# Autodesk Inventor assembly: 0.3rd Lawette - V3.0
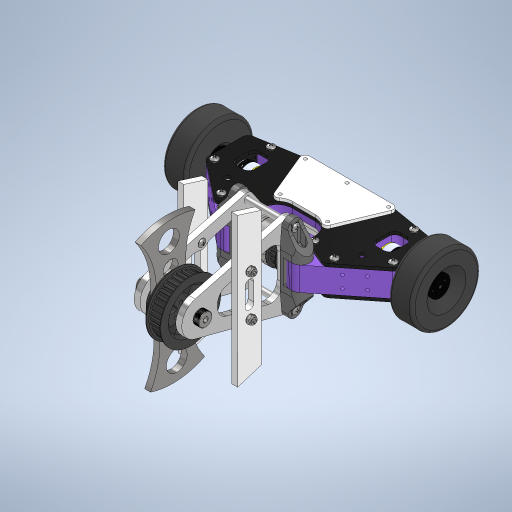
[picture p0: Inventor's stored thumbnail of the model, 512x512]
Saved by Autodesk Inventor 2023 (Build 270158000, 158)
## iProperties
Created: 2022-05-21
Part Number: 0.3rd Lawette - V3.0
Document SubType Name: Assembly
Designer: Nathan Cai
Mass: 1254.41 g
Surface Area: 3808.05 cm^2
Volume: 766.959 cm^3
Density: 1.63556 g/cm^3
Author: Nathan Cai
## Documents named in this file (23)
- E:\Documents\Inventor\0.3rd Lawette - V3.1\0.3rd Lawette - V3.1.iam
- E:\Documents\Inventor\0.3rd Lawette - V3.1\RR Brushless\RR-Brushless-Planetary.iam
- E:\Documents\Inventor\0.3rd Lawette - V3.1\Tattu 4S 650mah\Tattu 650mah 4S.iam
- E:\Documents\Inventor\0.3rd Lawette - V3.1\BL20A.ipt
- E:\Documents\Inventor\0.3rd Lawette - V3.1\Talon 25A ESC.ipt
- E:\Documents\Inventor\0.3rd Lawette - V3.1\Receiver (FrSky RX6R).ipt
- E:\Documents\Inventor\0.3rd Lawette - V3.1\Fingertech Power Switch\Fingertech Mini Power Switch.iam
- E:\Documents\Inventor\0.3rd Lawette - V3.1\Weapon Assembly.iam
- E:\Documents\Inventor\0.3rd Lawette - V3.1\Hubs (Fingertech Twisthub).ipt
- E:\Documents\Inventor\0.3rd Lawette - V3.1\Chassis.ipt
- E:\Documents\Inventor\0.3rd Lawette - V3.1\Tires (Fingertech Foam Wheels).ipt
- E:\Documents\Inventor\0.3rd Lawette - V3.1\Standoff 1.5in.ipt
- E:\Documents\Inventor\0.3rd Lawette - V3.1\Bracket.ipt
- E:\Documents\Inventor\Content Center Files\R2022\en-US\ANSI B18.6.3(27)\ANSI B18.6.3 - 6-32 UNC - 0.625(11).ipt
- E:\Documents\Inventor\0.3rd Lawette - V3.1\Motor Plates.ipt
- E:\Documents\Inventor\0.3rd Lawette - V3.1\Motor Plates - Rear Insert.ipt
- E:\Documents\Inventor\0.3rd Lawette - V3.1\Cover (Inner Bottom).ipt
- E:\Documents\Inventor\0.3rd Lawette - V3.1\Cover (Inner Top).ipt
- E:\Documents\Inventor\0.3rd Lawette - V3.1\Cover (Outer).ipt
- E:\Documents\Inventor\0.3rd Lawette - V3.1\Standoff 1in.ipt
- E:\Documents\Inventor\Content Center Files\R2022\en-US\ANSI B18.6.3(27)\ANSI B18.6.3 - 6-32 UNC - 0.875(11).ipt
- E:\Documents\Inventor\Content Center Files\R2022\en-US\ANSI B18.22.1\ANSI B18.22.1 - No. 6 - narrow - Type B.ipt
- E:\Documents\Inventor\Content Center Files\R2022\en-US\ANSI B18.6.3(27)\ANSI B18.6.3 - 6-32 UNC - 0.5(11).ipt
## Components (84 placed, 22 different names)
1. RR-Brushless-Planetary:1 [sub-assembly] — Mate:1, Mate:4, Mate:7, Flush:4, Mate:27, Mate:147
2. RR-Brushless-Planetary:2 [sub-assembly] — Mate:1, Mate:5, Mate:6, Flush:5, Mate:149
3. Tattu 650mah 4S:1 [sub-assembly] — Mate:15, Flush:9
4. BL20A:1 — Mate:2, Flush:1, Flush:2, Mate:14, Flush:7
5. BL20A:2 — Mate:2, Flush:1, Flush:2, Mate:3, Flush:3, Flush:8
6. Talon 25A ESC:1 — Mate:13, Flush:6, Mate:151
7. Receiver (FrSky RX6R):1 — Mate:3, Flush:3, Flush:8
8. Fingertech Mini Power Switch:1 [sub-assembly] — Flush:12, Mate:26, Mate:150
9. Hubs (Fingertech Twisthub):1 — Mate:4, Mate:7, Mate:8, Mate:11
10. Hubs (Fingertech Twisthub):2 — Mate:5, Mate:6, Mate:9, Mate:155
11. Chassis:1 — Flush:4, Flush:5, Mate:13, Flush:6, Mate:14, Flush:7, Mate:15, Flush:9, Flush:12, Mate:26, Mate:27, Mate:113, Mate:114, Mate:115, Mate:116, Mate:117, Mate:118, Mate:119, Mate:120, Mate:121, Mate:146, Flush:20, Mate:148, Flush:21, Mate:150, Mate:151, Mate:152, Mate:156, Mate:165, Mate:166, Mate:167, Mate:168, Mate:169, Mate:170, Mate:171, Mate:172, Mate:173, Mate:174, Mate:175, Mate:176, Mate:177, Flush:32, Mate:184, Mate:186, Mate:187
12. Tires (Fingertech Foam Wheels):1 — Mate:9, Mate:155
13. Tires (Fingertech Foam Wheels):2 — Mate:8, Mate:11
14. Motor Plates:1 — Mate:113, Mate:114, Mate:115
15. Motor Plates:2 — Mate:116, Mate:117, Mate:118
16. Motor Plates - Rear Insert:1 — Mate:146, Mate:147, Flush:20
17. Motor Plates - Rear Insert:2 — Mate:148, Mate:149, Flush:21
18. Cover (Inner Bottom):1 — Mate:152, Mate:159, Mate:160, Mate:161, Mate:216, Mate:217, Mate:218, Mate:219, Mate:220, Mate:221, Mate:222, Mate:223, Mate:224, Mate:225, Mate:226, Mate:227, Mate:228, Mate:229, Mate:230, Mate:231
19. Cover (Inner Top):1 — Mate:156, Mate:162, Mate:163, Mate:164, Mate:165, Mate:166, Mate:200, Mate:201, Mate:202, Mate:203, Mate:204, Mate:205, Mate:206, Mate:207, Mate:208, Mate:209, Mate:210, Mate:211, Mate:212, Mate:213, Mate:214, Mate:215
20. Cover (Outer):1 — Mate:159, Mate:160, Mate:161
21. Cover (Outer):2 — Mate:162, Mate:163, Mate:164
22. Standoff 1in:1 — Flush:22, Flush:23, Flush:24, Flush:25, Flush:26, Flush:27, Flush:28, Flush:29, Flush:30, Flush:31, Mate:167, Flush:32, Flush:33, Flush:34
23. Standoff 1in:2 — Flush:22, Mate:168
24. Standoff 1in:3 — Flush:25, Mate:175
25. Standoff 1in:4 — Flush:27, Mate:174
26. Standoff 1in:5 — Flush:29, Mate:173
27. Standoff 1in:6 — Flush:23, Mate:177
28. Standoff 1in:7 — Flush:24, Mate:176
29. Standoff 1in:8 — Flush:26, Mate:169
30. Standoff 1in:9 — Flush:28, Mate:170
31. Standoff 1in:10 — Flush:30, Mate:171
32. Standoff 1in:11 — Flush:31, Mate:172
33. Bracket:1 — Mate:178, Mate:179, Mate:180, Mate:185, Mate:196, Mate:197, Mate:198, Mate:199
34. Bracket:2 — Mate:181, Mate:182, Mate:183, Mate:184, Mate:192, Mate:193, Mate:194, Mate:195
35. Standoff 1in:12 — Mate:186, Flush:34
36. Standoff 1in:13 — Mate:187, Flush:33
37. Cross Recessed Truss Head Machine Screw - Type I - Inch No. 6 - 32 - 7/8:1 — Insert:5
38. Plain Washer (Inch) No. 6 - narrow - Type B:1 — Mate:192, Mate:193, Insert:3
39. Cross Recessed Truss Head Machine Screw - Type I - Inch No. 6 - 32 - 7/8:3 — Insert:3
40. Plain Washer (Inch) No. 6 - narrow - Type B:2 — Mate:194, Mate:195, Insert:4
41. Cross Recessed Truss Head Machine Screw - Type I - Inch No. 6 - 32 - 7/8:4 — Insert:4
42. Plain Washer (Inch) No. 6 - narrow - Type B:3 — Mate:196, Mate:197, Insert:5
43. Plain Washer (Inch) No. 6 - narrow - Type B:4 — Mate:198, Mate:199, Insert:6
44. Cross Recessed Truss Head Machine Screw - Type I - Inch No. 6 - 32 - 7/8:5 — Insert:6
45. Plain Washer (Inch) No. 6 - narrow - Type B:5 — Mate:200, Mate:201, Insert:7
46. Cross Recessed Truss Head Machine Screw - Type I - Inch No. 6 - 32 - 1/2:1 — Insert:7
47. Plain Washer (Inch) No. 6 - narrow - Type B:6 — Mate:202, Mate:203, Insert:8
48. Plain Washer (Inch) No. 6 - narrow - Type B:7 — Mate:204, Mate:205, Insert:9
49. Plain Washer (Inch) No. 6 - narrow - Type B:8 — Mate:206, Mate:207, Insert:10
50. Plain Washer (Inch) No. 6 - narrow - Type B:9 — Mate:208, Mate:209, Insert:11
51. Plain Washer (Inch) No. 6 - narrow - Type B:10 — Mate:210, Mate:211, Insert:12
52. Plain Washer (Inch) No. 6 - narrow - Type B:11 — Mate:212, Mate:213, Insert:13
53. Plain Washer (Inch) No. 6 - narrow - Type B:12 — Mate:214, Mate:215, Insert:14
54. Cross Recessed Truss Head Machine Screw - Type I - Inch No. 6 - 32 - 1/2:2 — Insert:8
55. Cross Recessed Truss Head Machine Screw - Type I - Inch No. 6 - 32 - 1/2:3 — Insert:9
56. Cross Recessed Truss Head Machine Screw - Type I - Inch No. 6 - 32 - 1/2:4 — Insert:10
57. Cross Recessed Truss Head Machine Screw - Type I - Inch No. 6 - 32 - 1/2:5 — Insert:11
58. Cross Recessed Truss Head Machine Screw - Type I - Inch No. 6 - 32 - 1/2:6 — Insert:12
59. Cross Recessed Truss Head Machine Screw - Type I - Inch No. 6 - 32 - 1/2:7 — Insert:13
60. Cross Recessed Truss Head Machine Screw - Type I - Inch No. 6 - 32 - 1/2:8 — Insert:14
61. Plain Washer (Inch) No. 6 - narrow - Type B:13 — Mate:216, Mate:217, Insert:15
62. Cross Recessed Truss Head Machine Screw - Type I - Inch No. 6 - 32 - 1/2:9 — Insert:15
63. Plain Washer (Inch) No. 6 - narrow - Type B:14 — Mate:218, Mate:219, Insert:16
64. Plain Washer (Inch) No. 6 - narrow - Type B:15 — Mate:220, Mate:221, Insert:17
65. Plain Washer (Inch) No. 6 - narrow - Type B:16 — Mate:222, Mate:223, Insert:18
66. Plain Washer (Inch) No. 6 - narrow - Type B:17 — Mate:224, Mate:225, Insert:19
67. Plain Washer (Inch) No. 6 - narrow - Type B:18 — Mate:226, Mate:227, Insert:20
68. Plain Washer (Inch) No. 6 - narrow - Type B:19 — Mate:228, Mate:229, Insert:21
69. Plain Washer (Inch) No. 6 - narrow - Type B:20 — Mate:230, Mate:231, Insert:22
70. Cross Recessed Truss Head Machine Screw - Type I - Inch No. 6 - 32 - 1/2:10 — Insert:16
71. Cross Recessed Truss Head Machine Screw - Type I - Inch No. 6 - 32 - 1/2:11 — Insert:17
72. Cross Recessed Truss Head Machine Screw - Type I - Inch No. 6 - 32 - 1/2:12 — Insert:18
73. Cross Recessed Truss Head Machine Screw - Type I - Inch No. 6 - 32 - 1/2:13 — Insert:19
74. Cross Recessed Truss Head Machine Screw - Type I - Inch No. 6 - 32 - 1/2:14 — Insert:20
75. Cross Recessed Truss Head Machine Screw - Type I - Inch No. 6 - 32 - 1/2:15 — Insert:21
76. Cross Recessed Truss Head Machine Screw - Type I - Inch No. 6 - 32 - 1/2:16 — Insert:22
77. Standoff 1.5in:7 — Mate:93, Mate:94, Mate:95, Mate:96, Mate:185
78. Standoff 1.5in:8 — Mate:97, Mate:98, Mate:99, Mate:100
79. Weapon Assembly:1 [sub-assembly] — Mate:178, Mate:179, Mate:180, Mate:181, Mate:182, Mate:183
80. Cross Recessed Truss Head Machine Screw - Type I - Inch No. 6 - 32 - 5/8:1 — Mate:93, Mate:94
81. Cross Recessed Truss Head Machine Screw - Type I - Inch No. 6 - 32 - 5/8:2 — Mate:95, Mate:96
82. Cross Recessed Truss Head Machine Screw - Type I - Inch No. 6 - 32 - 5/8:4 — Mate:99, Mate:100
83. Cross Recessed Truss Head Machine Screw - Type I - Inch No. 6 - 32 - 5/8:3 — Mate:97, Mate:98
84. Weapon Assembly:2 [sub-assembly] — Mate:119, Mate:120, Mate:121
## Relationships (159: Mate 112, Flush 27, Insert 20)
- Mate:1: RR-Brushless-Planetary:1 ↔ RR-Brushless-Planetary:2
- Mate:2: BL20A:1 ↔ BL20A:2
- Flush:1: BL20A:1 ↔ BL20A:2
- Flush:2: BL20A:1 ↔ BL20A:2
- Mate:3: BL20A:2 ↔ Receiver (FrSky RX6R):1
- Flush:3: BL20A:2 ↔ Receiver (FrSky RX6R):1
- Mate:4: RR-Brushless-Planetary:1 ↔ Hubs (Fingertech Twisthub):1
- Mate:5: RR-Brushless-Planetary:2 ↔ Hubs (Fingertech Twisthub):2
- Mate:6: RR-Brushless-Planetary:2 ↔ Hubs (Fingertech Twisthub):2
- Mate:7: RR-Brushless-Planetary:1 ↔ Hubs (Fingertech Twisthub):1
- Mate:8: Hubs (Fingertech Twisthub):1 ↔ Tires (Fingertech Foam Wheels):2
- Mate:9: Hubs (Fingertech Twisthub):2 ↔ Tires (Fingertech Foam Wheels):1
- Mate:11: Hubs (Fingertech Twisthub):1 ↔ Tires (Fingertech Foam Wheels):2
- Flush:4: RR-Brushless-Planetary:1 ↔ Chassis:1
- Flush:5: RR-Brushless-Planetary:2 ↔ Chassis:1
- Mate:13: Talon 25A ESC:1 ↔ Chassis:1
- Flush:6: Talon 25A ESC:1 ↔ Chassis:1
- Mate:14: BL20A:1 ↔ Chassis:1
- Flush:7: BL20A:1 ↔ Chassis:1
- Flush:8: BL20A:2 ↔ Receiver (FrSky RX6R):1
- Mate:15 (3.175 mm): Tattu 650mah 4S:1 ↔ Chassis:1
- Flush:9: Tattu 650mah 4S:1 ↔ Chassis:1
- Flush:12: Fingertech Mini Power Switch:1 ↔ Chassis:1
- [Mate]: Chassis:1 ↔ Standoff 1.5in:8
- [Mate]: Chassis:1 ↔ Standoff 1.5in:7
- Mate:26: Fingertech Mini Power Switch:1 ↔ Chassis:1
- Mate:27: RR-Brushless-Planetary:1 ↔ Chassis:1
- [Flush] (-6.35 mm): Chassis:1 ↔ Standoff 1.5in:8
- [Flush]: Standoff 1.5in:7 ↔ Standoff 1.5in:8
- Mate:93: Standoff 1.5in:7 ↔ Cross Recessed Truss Head Machine Screw - Type I - Inch No. 6 - 32 - 5/8:1
- Mate:94: Standoff 1.5in:7 ↔ Cross Recessed Truss Head Machine Screw - Type I - Inch No. 6 - 32 - 5/8:1
- Mate:95: Standoff 1.5in:7 ↔ Cross Recessed Truss Head Machine Screw - Type I - Inch No. 6 - 32 - 5/8:2
- Mate:96: Standoff 1.5in:7 ↔ Cross Recessed Truss Head Machine Screw - Type I - Inch No. 6 - 32 - 5/8:2
- Mate:97: Standoff 1.5in:8 ↔ Cross Recessed Truss Head Machine Screw - Type I - Inch No. 6 - 32 - 5/8:3
- Mate:98: Standoff 1.5in:8 ↔ Cross Recessed Truss Head Machine Screw - Type I - Inch No. 6 - 32 - 5/8:3
- Mate:99: Standoff 1.5in:8 ↔ Cross Recessed Truss Head Machine Screw - Type I - Inch No. 6 - 32 - 5/8:4
- Mate:100: Standoff 1.5in:8 ↔ Cross Recessed Truss Head Machine Screw - Type I - Inch No. 6 - 32 - 5/8:4
- Mate:113: Chassis:1 ↔ Motor Plates:1
- Mate:114: Chassis:1 ↔ Motor Plates:1
- Mate:115: Chassis:1 ↔ Motor Plates:1
- Mate:116: Chassis:1 ↔ Motor Plates:2
- Mate:117: Chassis:1 ↔ Motor Plates:2
- Mate:118: Chassis:1 ↔ Motor Plates:2
- Mate:119: Chassis:1 ↔ Weapon Assembly:2
- Mate:120: Chassis:1 ↔ Weapon Assembly:2
- Mate:121 (9.525 mm): Chassis:1 ↔ Weapon Assembly:2
- Mate:146: Chassis:1 ↔ Motor Plates - Rear Insert:1
- Mate:147: RR-Brushless-Planetary:1 ↔ Motor Plates - Rear Insert:1
- Flush:20: Chassis:1 ↔ Motor Plates - Rear Insert:1
- Mate:148: Chassis:1 ↔ Motor Plates - Rear Insert:2
- Mate:149: RR-Brushless-Planetary:2 ↔ Motor Plates - Rear Insert:2
- Flush:21: Chassis:1 ↔ Motor Plates - Rear Insert:2
- Mate:150: Fingertech Mini Power Switch:1 ↔ Chassis:1
- Mate:151: Talon 25A ESC:1 ↔ Chassis:1
- Mate:152: Chassis:1 ↔ Cover (Inner Bottom):1
- Mate:155: Hubs (Fingertech Twisthub):2 ↔ Tires (Fingertech Foam Wheels):1
- Mate:156: Chassis:1 ↔ Cover (Inner Top):1
- Mate:159: Cover (Inner Bottom):1 ↔ Cover (Outer):1
- Mate:160: Cover (Inner Bottom):1 ↔ Cover (Outer):1
- Mate:161: Cover (Inner Bottom):1 ↔ Cover (Outer):1
- Mate:162: Cover (Inner Top):1 ↔ Cover (Outer):2
- Mate:163: Cover (Inner Top):1 ↔ Cover (Outer):2
- Mate:164: Cover (Inner Top):1 ↔ Cover (Outer):2
- Mate:165: Chassis:1 ↔ Cover (Inner Top):1
- Mate:166: Chassis:1 ↔ Cover (Inner Top):1
- Flush:22: Standoff 1in:1 ↔ Standoff 1in:2
- Flush:23: Standoff 1in:1 ↔ Standoff 1in:6
- Flush:24: Standoff 1in:1 ↔ Standoff 1in:7
- Flush:25: Standoff 1in:1 ↔ Standoff 1in:3
- Flush:26: Standoff 1in:1 ↔ Standoff 1in:8
- Flush:27: Standoff 1in:1 ↔ Standoff 1in:4
- Flush:28: Standoff 1in:1 ↔ Standoff 1in:9
- Flush:29: Standoff 1in:1 ↔ Standoff 1in:5
- Flush:30: Standoff 1in:1 ↔ Standoff 1in:10
- Flush:31: Standoff 1in:1 ↔ Standoff 1in:11
- Mate:167: Chassis:1 ↔ Standoff 1in:1
- Mate:168: Chassis:1 ↔ Standoff 1in:2
- Mate:169: Chassis:1 ↔ Standoff 1in:8
- Mate:170: Chassis:1 ↔ Standoff 1in:9
- Mate:171: Chassis:1 ↔ Standoff 1in:10
- Mate:172: Chassis:1 ↔ Standoff 1in:11
- Mate:173: Chassis:1 ↔ Standoff 1in:5
- Mate:174: Chassis:1 ↔ Standoff 1in:4
- Mate:175: Chassis:1 ↔ Standoff 1in:3
- Mate:176: Chassis:1 ↔ Standoff 1in:7
- Mate:177: Chassis:1 ↔ Standoff 1in:6
- Flush:32: Chassis:1 ↔ Standoff 1in:1
- Mate:178: Bracket:1 ↔ Weapon Assembly:1
- Mate:179: Bracket:1 ↔ Weapon Assembly:1
- Mate:180: Bracket:1 ↔ Weapon Assembly:1
- Mate:181: Bracket:2 ↔ Weapon Assembly:1
- Mate:182: Bracket:2 ↔ Weapon Assembly:1
- Mate:183: Bracket:2 ↔ Weapon Assembly:1
- Mate:184: Chassis:1 ↔ Bracket:2
- Mate:185: Bracket:1 ↔ Standoff 1.5in:7
- Mate:186: Chassis:1 ↔ Standoff 1in:12
- Mate:187: Chassis:1 ↔ Standoff 1in:13
- Flush:33: Standoff 1in:1 ↔ Standoff 1in:13
- Flush:34: Standoff 1in:1 ↔ Standoff 1in:12
- Mate:192: Bracket:2 ↔ Plain Washer (Inch) No. 6 - narrow - Type B:1
- Mate:193: Bracket:2 ↔ Plain Washer (Inch) No. 6 - narrow - Type B:1
- Mate:194: Bracket:2 ↔ Plain Washer (Inch) No. 6 - narrow - Type B:2
- Mate:195: Bracket:2 ↔ Plain Washer (Inch) No. 6 - narrow - Type B:2
- Insert:3: Plain Washer (Inch) No. 6 - narrow - Type B:1 ↔ Cross Recessed Truss Head Machine Screw - Type I - Inch No. 6 - 32 - 7/8:3
- Insert:4: Plain Washer (Inch) No. 6 - narrow - Type B:2 ↔ Cross Recessed Truss Head Machine Screw - Type I - Inch No. 6 - 32 - 7/8:4
- Mate:196: Bracket:1 ↔ Plain Washer (Inch) No. 6 - narrow - Type B:3
- Mate:197: Bracket:1 ↔ Plain Washer (Inch) No. 6 - narrow - Type B:3
- Mate:198: Bracket:1 ↔ Plain Washer (Inch) No. 6 - narrow - Type B:4
- Mate:199: Bracket:1 ↔ Plain Washer (Inch) No. 6 - narrow - Type B:4
- Insert:5: Cross Recessed Truss Head Machine Screw - Type I - Inch No. 6 - 32 - 7/8:1 ↔ Plain Washer (Inch) No. 6 - narrow - Type B:3
- Insert:6: Plain Washer (Inch) No. 6 - narrow - Type B:4 ↔ Cross Recessed Truss Head Machine Screw - Type I - Inch No. 6 - 32 - 7/8:5
- Mate:200: Cover (Inner Top):1 ↔ Plain Washer (Inch) No. 6 - narrow - Type B:5
- Mate:201: Cover (Inner Top):1 ↔ Plain Washer (Inch) No. 6 - narrow - Type B:5
- Mate:202: Cover (Inner Top):1 ↔ Plain Washer (Inch) No. 6 - narrow - Type B:6
- Mate:203: Cover (Inner Top):1 ↔ Plain Washer (Inch) No. 6 - narrow - Type B:6
- Mate:204: Cover (Inner Top):1 ↔ Plain Washer (Inch) No. 6 - narrow - Type B:7
- Mate:205: Cover (Inner Top):1 ↔ Plain Washer (Inch) No. 6 - narrow - Type B:7
- Mate:206: Cover (Inner Top):1 ↔ Plain Washer (Inch) No. 6 - narrow - Type B:8
- Mate:207: Cover (Inner Top):1 ↔ Plain Washer (Inch) No. 6 - narrow - Type B:8
- Mate:208: Cover (Inner Top):1 ↔ Plain Washer (Inch) No. 6 - narrow - Type B:9
- Mate:209: Cover (Inner Top):1 ↔ Plain Washer (Inch) No. 6 - narrow - Type B:9
- Mate:210: Cover (Inner Top):1 ↔ Plain Washer (Inch) No. 6 - narrow - Type B:10
- Mate:211: Cover (Inner Top):1 ↔ Plain Washer (Inch) No. 6 - narrow - Type B:10
- Mate:212: Cover (Inner Top):1 ↔ Plain Washer (Inch) No. 6 - narrow - Type B:11
- Mate:213: Cover (Inner Top):1 ↔ Plain Washer (Inch) No. 6 - narrow - Type B:11
- Mate:214: Cover (Inner Top):1 ↔ Plain Washer (Inch) No. 6 - narrow - Type B:12
- Mate:215: Cover (Inner Top):1 ↔ Plain Washer (Inch) No. 6 - narrow - Type B:12
- Insert:7: Plain Washer (Inch) No. 6 - narrow - Type B:5 ↔ Cross Recessed Truss Head Machine Screw - Type I - Inch No. 6 - 32 - 1/2:1
- Insert:8: Plain Washer (Inch) No. 6 - narrow - Type B:6 ↔ Cross Recessed Truss Head Machine Screw - Type I - Inch No. 6 - 32 - 1/2:2
- Insert:9: Plain Washer (Inch) No. 6 - narrow - Type B:7 ↔ Cross Recessed Truss Head Machine Screw - Type I - Inch No. 6 - 32 - 1/2:3
- Insert:10: Plain Washer (Inch) No. 6 - narrow - Type B:8 ↔ Cross Recessed Truss Head Machine Screw - Type I - Inch No. 6 - 32 - 1/2:4
- Insert:11: Plain Washer (Inch) No. 6 - narrow - Type B:9 ↔ Cross Recessed Truss Head Machine Screw - Type I - Inch No. 6 - 32 - 1/2:5
- Insert:12: Plain Washer (Inch) No. 6 - narrow - Type B:10 ↔ Cross Recessed Truss Head Machine Screw - Type I - Inch No. 6 - 32 - 1/2:6
- Insert:13: Plain Washer (Inch) No. 6 - narrow - Type B:11 ↔ Cross Recessed Truss Head Machine Screw - Type I - Inch No. 6 - 32 - 1/2:7
- Insert:14: Plain Washer (Inch) No. 6 - narrow - Type B:12 ↔ Cross Recessed Truss Head Machine Screw - Type I - Inch No. 6 - 32 - 1/2:8
- Mate:216: Cover (Inner Bottom):1 ↔ Plain Washer (Inch) No. 6 - narrow - Type B:13
- Mate:217: Cover (Inner Bottom):1 ↔ Plain Washer (Inch) No. 6 - narrow - Type B:13
- Mate:218: Cover (Inner Bottom):1 ↔ Plain Washer (Inch) No. 6 - narrow - Type B:14
- Mate:219: Cover (Inner Bottom):1 ↔ Plain Washer (Inch) No. 6 - narrow - Type B:14
- Mate:220: Cover (Inner Bottom):1 ↔ Plain Washer (Inch) No. 6 - narrow - Type B:15
- Mate:221: Cover (Inner Bottom):1 ↔ Plain Washer (Inch) No. 6 - narrow - Type B:15
- Mate:222: Cover (Inner Bottom):1 ↔ Plain Washer (Inch) No. 6 - narrow - Type B:16
- Mate:223: Cover (Inner Bottom):1 ↔ Plain Washer (Inch) No. 6 - narrow - Type B:16
- Mate:224: Cover (Inner Bottom):1 ↔ Plain Washer (Inch) No. 6 - narrow - Type B:17
- Mate:225: Cover (Inner Bottom):1 ↔ Plain Washer (Inch) No. 6 - narrow - Type B:17
- Mate:226: Cover (Inner Bottom):1 ↔ Plain Washer (Inch) No. 6 - narrow - Type B:18
- Mate:227: Cover (Inner Bottom):1 ↔ Plain Washer (Inch) No. 6 - narrow - Type B:18
- Mate:228: Cover (Inner Bottom):1 ↔ Plain Washer (Inch) No. 6 - narrow - Type B:19
- Mate:229: Cover (Inner Bottom):1 ↔ Plain Washer (Inch) No. 6 - narrow - Type B:19
- Mate:230: Cover (Inner Bottom):1 ↔ Plain Washer (Inch) No. 6 - narrow - Type B:20
- Mate:231: Cover (Inner Bottom):1 ↔ Plain Washer (Inch) No. 6 - narrow - Type B:20
- Insert:15: Plain Washer (Inch) No. 6 - narrow - Type B:13 ↔ Cross Recessed Truss Head Machine Screw - Type I - Inch No. 6 - 32 - 1/2:9
- Insert:16: Plain Washer (Inch) No. 6 - narrow - Type B:14 ↔ Cross Recessed Truss Head Machine Screw - Type I - Inch No. 6 - 32 - 1/2:10
- Insert:17: Plain Washer (Inch) No. 6 - narrow - Type B:15 ↔ Cross Recessed Truss Head Machine Screw - Type I - Inch No. 6 - 32 - 1/2:11
- Insert:18: Plain Washer (Inch) No. 6 - narrow - Type B:16 ↔ Cross Recessed Truss Head Machine Screw - Type I - Inch No. 6 - 32 - 1/2:12
- Insert:19: Plain Washer (Inch) No. 6 - narrow - Type B:17 ↔ Cross Recessed Truss Head Machine Screw - Type I - Inch No. 6 - 32 - 1/2:13
- Insert:20: Plain Washer (Inch) No. 6 - narrow - Type B:18 ↔ Cross Recessed Truss Head Machine Screw - Type I - Inch No. 6 - 32 - 1/2:14
- Insert:21: Plain Washer (Inch) No. 6 - narrow - Type B:19 ↔ Cross Recessed Truss Head Machine Screw - Type I - Inch No. 6 - 32 - 1/2:15
- Insert:22: Plain Washer (Inch) No. 6 - narrow - Type B:20 ↔ Cross Recessed Truss Head Machine Screw - Type I - Inch No. 6 - 32 - 1/2:16
